# Autodesk Inventor assembly: Pata - Ensamble 3 DOF
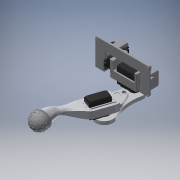
[picture p0: Inventor's stored thumbnail of the model, 180x180]
Saved by Autodesk Inventor 2019 (Build 230136000, 136)
## iProperties
Created: 2020-03-08
Part Number: Pata - Ensamble 3 DOF
Material: Genérico
Document SubType Name: Assembly
Designer: eddysanoli
Author: eddysanoli
## Documents named in this file (8)
- E:\Escritorio\Temporal\Documentos\Robótica I\Robótica I - Proyecto Cuadrúpedo\Pata - Ensamble 3 DOF.iam
- E:\Escritorio\Temporal\Documentos\Robótica I\Robótica I - Proyecto Cuadrúpedo\Servo MG996R\Servo MG996R - Ensamble - Sin Flor.iam
- E:\Escritorio\Temporal\Documentos\Robótica I\Robótica I - Proyecto Cuadrúpedo\Pata - Antebrazo.ipt
- E:\Escritorio\Temporal\Documentos\Robótica I\Robótica I - Proyecto Cuadrúpedo\Servo MG996R\TowerPro SG5010 - Acople Hélice.ipt
- E:\Escritorio\Temporal\Documentos\Robótica I\Robótica I - Proyecto Cuadrúpedo\Pata - Brazo - Pata Ninjaflex.ipt
- E:\Escritorio\Temporal\Documentos\Robótica I\Robótica I - Proyecto Cuadrúpedo\Pata - Pie - Textura.ipt
- E:\Escritorio\Temporal\Documentos\Robótica I\Robótica I - Proyecto Cuadrúpedo\Cuerpo - Acople Hombro.ipt
- E:\Escritorio\Temporal\Documentos\Robótica I\Robótica I - Proyecto Cuadrúpedo\Pata - Hombro.ipt
## Components (11 placed, 7 different names)
1. Servo MG996R - Ensamble - Sin Flor:1 [sub-assembly] — Coincidencia:19, Coincidencia:20, Coincidencia:21
2. Pata - Antebrazo:1
3. TowerPro SG5010 - Acople Hélice:1
4. TowerPro SG5010 - Acople Hélice:2
5. Servo MG996R - Ensamble - Sin Flor:2 [sub-assembly]
6. Pata - Brazo - Pata Ninjaflex:1
7. Pata - Pie - Textura:1
8. Cuerpo - Acople Hombro:1 — Coincidencia:14, Coincidencia:15, Coincidencia:16, Coincidencia:22
9. Servo MG996R - Ensamble - Sin Flor:3 [sub-assembly] — Coincidencia:14, Coincidencia:15, Coincidencia:16, Nivelación:3, Coincidencia:17
10. TowerPro SG5010 - Acople Hélice:3 — Nivelación:3, Coincidencia:17, Coincidencia:18
11. Pata - Hombro:1 — Coincidencia:18, Coincidencia:19, Coincidencia:20, Coincidencia:21, Coincidencia:22
## Relationships (25: Mate 22, Flush 3)
- [Mate]: Pata - Antebrazo:1 ↔ TowerPro SG5010 - Acople Hélice:2
- [Mate]: Pata - Antebrazo:1 ↔ TowerPro SG5010 - Acople Hélice:2
- [Mate]: Pata - Antebrazo:1 ↔ TowerPro SG5010 - Acople Hélice:2
- [Mate]: Pata - Antebrazo:1 ↔ TowerPro SG5010 - Acople Hélice:1
- [Mate]: Pata - Antebrazo:1 ↔ TowerPro SG5010 - Acople Hélice:1
- [Mate]: Pata - Antebrazo:1 ↔ TowerPro SG5010 - Acople Hélice:1
- [Flush]: Servo MG996R - Ensamble - Sin Flor:1 ↔ TowerPro SG5010 - Acople Hélice:2
- [Mate]: Servo MG996R - Ensamble - Sin Flor:1 ↔ TowerPro SG5010 - Acople Hélice:2
- [Mate]: Pata - Brazo - Pata Ninjaflex:1 ↔ Pata - Pie - Textura:1
- [Mate]: Pata - Brazo - Pata Ninjaflex:1 ↔ Pata - Pie - Textura:1
- [Mate]: Servo MG996R - Ensamble - Sin Flor:2 ↔ Pata - Brazo - Pata Ninjaflex:1
- [Mate]: Servo MG996R - Ensamble - Sin Flor:2 ↔ Pata - Brazo - Pata Ninjaflex:1
- [Mate]: Servo MG996R - Ensamble - Sin Flor:2 ↔ Pata - Brazo - Pata Ninjaflex:1
- [Flush]: TowerPro SG5010 - Acople Hélice:1 ↔ Servo MG996R - Ensamble - Sin Flor:2
- [Mate]: TowerPro SG5010 - Acople Hélice:1 ↔ Servo MG996R - Ensamble - Sin Flor:2
- Coincidencia:14 [Mate]: Cuerpo - Acople Hombro:1 ↔ Servo MG996R - Ensamble - Sin Flor:3
- Coincidencia:15 [Mate]: Cuerpo - Acople Hombro:1 ↔ Servo MG996R - Ensamble - Sin Flor:3
- Coincidencia:16 [Mate]: Cuerpo - Acople Hombro:1 ↔ Servo MG996R - Ensamble - Sin Flor:3
- Nivelación:3 [Flush]: Servo MG996R - Ensamble - Sin Flor:3 ↔ TowerPro SG5010 - Acople Hélice:3
- Coincidencia:17 [Mate]: Servo MG996R - Ensamble - Sin Flor:3 ↔ TowerPro SG5010 - Acople Hélice:3
- Coincidencia:18 [Mate]: TowerPro SG5010 - Acople Hélice:3 ↔ Pata - Hombro:1
- Coincidencia:19 [Mate]: Servo MG996R - Ensamble - Sin Flor:1 ↔ Pata - Hombro:1
- Coincidencia:20 [Mate]: Servo MG996R - Ensamble - Sin Flor:1 ↔ Pata - Hombro:1
- Coincidencia:21 [Mate]: Servo MG996R - Ensamble - Sin Flor:1 ↔ Pata - Hombro:1
- Coincidencia:22 [Mate]: Cuerpo - Acople Hombro:1 ↔ Pata - Hombro:1
## Named parameters: d98_d62 = 0 mm, d99_d63 = 0 mm
